# Autodesk Inventor assembly: AssemblySpring
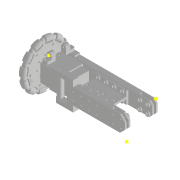
[picture p0: Inventor's stored thumbnail of the model, 180x180]
Saved by Autodesk Inventor 2022 (Build 260153000, 153)
## iProperties
Created: 2022-11-21
Part Number: AssemblySpring
Document SubType Name: Assembly
Designer: MVeszpremi
Author: MVeszpremi
## Documents named in this file (8)
- C:\Users\veszp\Dropbox\180DAB CAD\SpringLoadedDesign\AssemblySpring.iam
- C:\Users\veszp\Dropbox\180DAB CAD\SpringLoadedDesign\StepperMotorHolder_Spring.ipt
- C:\Users\veszp\Dropbox\180DAB CAD\SpringLoadedDesign\RobotBaseMotorExtUpper_Spring.ipt
- C:\Users\veszp\Dropbox\180DAB CAD\SpringLoadedDesign\RobotBaseMotorExtLower_Spring.ipt
- C:\Users\veszp\Dropbox\180DAB CAD\SpringLoadedDesign\SpringConn.ipt
- C:\Users\veszp\Dropbox\180DAB CAD\SpringLoadedDesign\ExtConnector_Spring.ipt
- C:\Users\veszp\Dropbox\180DAB CAD\Wheel.ipt
- C:\Users\veszp\Dropbox\180DAB CAD\gearedNema17.ipt
## Components (8 placed, 7 different names)
1. StepperMotorHolder_Spring:1 — Mate:9, Mate:10, Mate:16, Mate:17, Mate:18, Angle:2, Mate:20
2. RobotBaseMotorExtLower_Spring:1 — Mate:7, Mate:8, Mate:12, Mate:15, Mate:23
3. SpringConn:1 — Mate:7, Mate:8, Angle:1, Mate:11
4. SpringConn:2 — Mate:9, Mate:10, Angle:1, Mate:11
5. ExtConnector_Spring:1 — Mate:12, Mate:15, Mate:19, Mate:21, Mate:22, Mate:23
6. Wheel:1 — Mate:16, Mate:17
7. gearedNema17:1 — Mate:18, Angle:2
8. RobotBaseMotorExtUpper_Spring:1 — Mate:19, Mate:20, Mate:21, Mate:22
## Relationships (17: Mate 15, Angle 2)
- Mate:7: RobotBaseMotorExtLower_Spring:1 ↔ SpringConn:1
- Mate:8: RobotBaseMotorExtLower_Spring:1 ↔ SpringConn:1
- Mate:9: StepperMotorHolder_Spring:1 ↔ SpringConn:2
- Mate:10: StepperMotorHolder_Spring:1 ↔ SpringConn:2
- Angle:1 (180 deg): SpringConn:1 ↔ SpringConn:2
- Mate:11: SpringConn:1 ↔ SpringConn:2
- Mate:12: RobotBaseMotorExtLower_Spring:1 ↔ ExtConnector_Spring:1
- Mate:15: RobotBaseMotorExtLower_Spring:1 ↔ ExtConnector_Spring:1
- Mate:16: StepperMotorHolder_Spring:1 ↔ Wheel:1
- Mate:17 (10 mm): StepperMotorHolder_Spring:1 ↔ Wheel:1
- Mate:18: StepperMotorHolder_Spring:1 ↔ gearedNema17:1
- Angle:2 (0 deg): StepperMotorHolder_Spring:1 ↔ gearedNema17:1
- Mate:19: ExtConnector_Spring:1 ↔ RobotBaseMotorExtUpper_Spring:1
- Mate:20: StepperMotorHolder_Spring:1 ↔ RobotBaseMotorExtUpper_Spring:1
- Mate:21: ExtConnector_Spring:1 ↔ RobotBaseMotorExtUpper_Spring:1
- Mate:22: ExtConnector_Spring:1 ↔ RobotBaseMotorExtUpper_Spring:1
- Mate:23: RobotBaseMotorExtLower_Spring:1 ↔ ExtConnector_Spring:1
